# Autodesk Inventor assembly: RCP-2.0
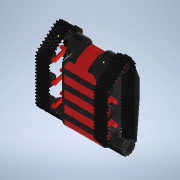
[picture p0: Inventor's stored thumbnail of the model, 180x180]
Saved by Autodesk Inventor 2020 (Build 240168000, 168)
## iProperties
Created: 2021-06-14
Part Number: RCP-2.0
Document SubType Name: Assembly
Designer: I_Love_U_Bogdan
Author: I_Love_U_Bogdan
## Documents named in this file (33)
- C:\Users\I_Love_U_Bogdan\Desktop\Work\Гусеничная платформа\RCP-2.0.iam
- C:\Users\I_Love_U_Bogdan\Desktop\Work\Гусеничная платформа\Корпус внутр.ipt
- C:\Users\I_Love_U_Bogdan\Desktop\Work\Гусеничная платформа\Корпус внутр2.ipt
- C:\Users\I_Love_U_Bogdan\Desktop\Work\Гусеничная платформа\Корпус.ipt
- C:\Users\I_Love_U_Bogdan\Desktop\Work\Гусеничная платформа\Корпус4.ipt
- C:\Users\I_Love_U_Bogdan\Desktop\Work\Гусеничная платформа\Перед-верх.ipt
- C:\Users\I_Love_U_Bogdan\Desktop\Work\Гусеничная платформа\СкреплениеКорпусПеред.ipt
- C:\Users\I_Love_U_Bogdan\Desktop\Work\Гусеничная платформа\РеброСкрепления.ipt
- C:\Users\I_Love_U_Bogdan\Desktop\Work\Гусеничная платформа\ВерхнийКрюк.ipt
- C:\Users\I_Love_U_Bogdan\Desktop\Work\Гусеничная платформа\РельсКрышки.ipt
- C:\Users\I_Love_U_Bogdan\Desktop\Work\Гусеничная платформа\Держатель каскада.ipt
- C:\Users\I_Love_U_Bogdan\Desktop\Work\Гусеничная платформа\запорные зубцы.ipt
- C:\Users\I_Love_U_Bogdan\Desktop\Work\Гусеничная платформа\Крышка.ipt
- C:\Users\I_Love_U_Bogdan\Desktop\Work\Гусеничная платформа\РучкаКрышки.ipt
- C:\Users\I_Love_U_Bogdan\Desktop\Work\Гусеничная платформа\Держатель каскада2.ipt
- C:\Users\I_Love_U_Bogdan\Desktop\Work\Гусеничная платформа\Пластина.ipt
- C:\Users\I_Love_U_Bogdan\Desktop\Work\Гусеничная платформа\ВедущееКолесо V2.ipt
- C:\Users\I_Love_U_Bogdan\Desktop\Work\Гусеничная платформа\Шаговик17.ipt
- C:\Users\I_Love_U_Bogdan\Desktop\Work\Гусеничная платформа\Муфта2.ipt
- C:\Users\I_Love_U_Bogdan\Desktop\Work\Гусеничная платформа\Втулка.ipt
- C:\Users\I_Love_U_Bogdan\Desktop\Work\Гусеничная платформа\ВнутрНат.ipt
- C:\Users\I_Love_U_Bogdan\Desktop\Work\Гусеничная платформа\ВнутрНатПр.ipt
- C:\Users\I_Love_U_Bogdan\Desktop\Work\Гусеничная платформа\ВнешНат.ipt
- C:\Users\I_Love_U_Bogdan\Desktop\Work\Гусеничная платформа\ВнешНатПр.ipt
- C:\Users\I_Love_U_Bogdan\Desktop\Work\Гусеничная платформа\ОпорныйКаток.ipt
- C:\Users\I_Love_U_Bogdan\Desktop\Work\Гусеничная платформа\ОпорныйКаток2.ipt
- C:\Users\I_Love_U_Bogdan\Desktop\Work\Гусеничная платформа\СкреплениеКатков.ipt
- C:\Users\I_Love_U_Bogdan\Desktop\Work\Гусеничная платформа\РычагОпорного.ipt
- C:\Users\I_Love_U_Bogdan\Desktop\Work\Гусеничная платформа\РычагОпорногоПравый.ipt
- C:\Users\I_Love_U_Bogdan\Desktop\Work\Гусеничная платформа\Надкрылок.ipt
- C:\Users\I_Love_U_Bogdan\Desktop\Work\Гусеничная платформа\НадкрылокПравый.ipt
- C:\Users\I_Love_U_Bogdan\Desktop\Work\Гусеничная платформа\Направляющая1.ipt
- C:\Users\I_Love_U_Bogdan\Desktop\Work\Гусеничная платформа\ТракV2.ipt
## Components (201 placed, 32 different names)
1. Шаговик17:1 — Совмещение:72, Совмещение:73, Совмещение:74, Совмещение:78, Совмещение:79
2. Шаговик17:2 — Совмещение:75, Совмещение:76, Совмещение:77, Совмещение:80, Совмещение:81
3. ВедущееКолесо V2:2 — Совмещение:82, Совмещение:86, Совмещение:87, Совмещение:195
4. Муфта2:1 — Совмещение:78, Совмещение:79, Совмещение:83, Совмещение:84, Совмещение:85, Угол:1
5. Муфта2:2 — Совмещение:80, Совмещение:81, Совмещение:82, Совмещение:86, Совмещение:87, Угол:2
6. ВедущееКолесо V2:3 — Совмещение:83, Совмещение:84, Совмещение:85, Совмещение:192
7. РычагОпорного:1 — Совмещение:116, Совмещение:117, Совмещение:128, Совмещение:171, Совмещение:175
8. РычагОпорного:2 — Совмещение:118, Совмещение:120, Совмещение:129, Совмещение:172, Совмещение:176
9. РычагОпорного:3 — Совмещение:119, Совмещение:121, Совмещение:130, Совмещение:173, Совмещение:177
10. РычагОпорногоПравый:1 — Совмещение:122, Совмещение:127, Совмещение:131, Совмещение:180, Совмещение:184
11. РычагОпорногоПравый:2 — Совмещение:123, Совмещение:126, Совмещение:132, Совмещение:179, Совмещение:183
12. РычагОпорногоПравый:3 — Совмещение:124, Совмещение:125, Совмещение:133, Совмещение:178, Совмещение:185
13. Надкрылок:1 — Совмещение:186, Совмещение:187, Совмещение:188
14. НадкрылокПравый:1 — Совмещение:189, Совмещение:190, Совмещение:191
15. Направляющая1:1 — Заподлицо:15, Заподлицо:16, Совмещение:194, Совмещение:196
16. Втулка:1 — Совмещение:91, Совмещение:92, Совмещение:93, Совмещение:95, Совмещение:99
17. Втулка:2 — Совмещение:88, Совмещение:89, Совмещение:90, Совмещение:94, Совмещение:98
18. ВнутрНат:1 — Совмещение:94, Совмещение:97, Совмещение:98, Совмещение:100, Совмещение:102
19. ВнутрНатПр:1 — Совмещение:95, Совмещение:96, Совмещение:99, Совмещение:101, Совмещение:103
20. ВнешНат:1 — Совмещение:100, Совмещение:102, Совмещение:170, Совмещение:174
21. ВнешНатПр:1 — Совмещение:101, Совмещение:103, Совмещение:181, Совмещение:182
22. ОпорныйКаток:1 — Совмещение:104, Совмещение:105, Совмещение:106, Совмещение:109
23. ОпорныйКаток2:1 — Совмещение:104, Совмещение:105, Совмещение:106, Совмещение:107, Совмещение:108, Совмещение:170, Совмещение:174
24. СкреплениеКатков:1 — Совмещение:107, Совмещение:108, Совмещение:109
25. ОпорныйКаток:2
26. ОпорныйКаток2:2 — Совмещение:171, Совмещение:175
27. СкреплениеКатков:2
28. ОпорныйКаток:3
29. ОпорныйКаток2:3 — Совмещение:172, Совмещение:176
30. СкреплениеКатков:3
31. ОпорныйКаток:4
32. ОпорныйКаток2:4 — Совмещение:173, Совмещение:177
33. СкреплениеКатков:4
34. ОпорныйКаток:5
35. ОпорныйКаток2:5 — Совмещение:178, Совмещение:185
36. СкреплениеКатков:5
37. ОпорныйКаток:6
38. ОпорныйКаток2:6 — Совмещение:179, Совмещение:183
39. СкреплениеКатков:6
40. ОпорныйКаток:7
41. ОпорныйКаток2:7 — Совмещение:180, Совмещение:184
42. СкреплениеКатков:7
43. ОпорныйКаток:8
44. ОпорныйКаток2:8 — Совмещение:181, Совмещение:182
45. СкреплениеКатков:8
46. Корпус внутр:1 — Совмещение:1, Совмещение:2, Совмещение:3, Совмещение:4, Заподлицо:1, Заподлицо:2, Совмещение:5, Заподлицо:3, Заподлицо:4, Совмещение:7, Заподлицо:7, Заподлицо:8, Совмещение:8, Совмещение:9, Совмещение:10
47. Корпус внутр2:1 — Совмещение:4, Заподлицо:1, Заподлицо:2, Совмещение:6, Заподлицо:5, Заподлицо:6, Совмещение:11, Совмещение:12, Совмещение:13, Совмещение:14, Совмещение:15, Совмещение:16, Совмещение:17, Совмещение:18, Совмещение:19, Совмещение:20
48. Корпус:1 — Совмещение:5, Заподлицо:3, Заподлицо:4, Совмещение:34, Совмещение:35, Совмещение:36, Заподлицо:13, Совмещение:71, Совмещение:72, Совмещение:73, Совмещение:74, Совмещение:88, Совмещение:89, Совмещение:90, Совмещение:97, Совмещение:116, Совмещение:117, Совмещение:118, Совмещение:119, Совмещение:120, Совмещение:121, Совмещение:128, Совмещение:129, Совмещение:130, Совмещение:186, Совмещение:187, Совмещение:188, Заподлицо:15, Заподлицо:16, Угол:1
49. Корпус4:1 — Совмещение:6, Заподлицо:5, Заподлицо:6, Совмещение:21, Совмещение:22, Совмещение:23, Совмещение:24, Совмещение:25, Совмещение:37, Совмещение:38, Совмещение:39, Совмещение:75, Совмещение:76, Совмещение:77, Совмещение:91, Совмещение:92, Совмещение:93, Совмещение:96, Совмещение:122, Совмещение:123, Совмещение:124, Совмещение:125, Совмещение:126, Совмещение:127, Совмещение:131, Совмещение:132, Совмещение:133, Совмещение:189, Совмещение:190, Совмещение:191, Угол:2
50. Перед-верх:1 — Совмещение:7, Заподлицо:7, Заподлицо:8, Совмещение:26, Совмещение:27, Совмещение:28, Совмещение:29, Совмещение:30, Совмещение:31, Совмещение:32, Совмещение:33, Заподлицо:9, Заподлицо:10, Заподлицо:11, Заподлицо:12, Заподлицо:14
51. СкреплениеКорпусПеред:1 — Совмещение:8, Совмещение:9, Совмещение:10
52. РеброСкрепления:1 — Совмещение:14, Совмещение:17, Совмещение:22
53. РеброСкрепления:2 — Совмещение:13, Совмещение:18, Совмещение:23
54. РеброСкрепления:3 — Совмещение:12, Совмещение:19, Совмещение:24
55. РеброСкрепления:4 — Совмещение:11, Совмещение:20, Совмещение:25
56. РеброСкрепления:5 — Совмещение:15, Совмещение:16, Совмещение:21
57. ВерхнийКрюк:1 — Совмещение:32, Совмещение:33, Заподлицо:9
58. ВерхнийКрюк:2 — Совмещение:28, Совмещение:29, Заподлицо:11
59. ВерхнийКрюк:3 — Совмещение:30, Совмещение:31, Заподлицо:10
60. ВерхнийКрюк:4 — Совмещение:26, Совмещение:27, Заподлицо:12
61. РельсКрышки:1 — Совмещение:34, Совмещение:35, Совмещение:36
62. РельсКрышки:2 — Совмещение:37, Совмещение:38, Совмещение:39
63. Держатель каскада:1 — Совмещение:43, Совмещение:44, Совмещение:45, Совмещение:48
64. запорные зубцы:1 — Совмещение:40, Совмещение:41, Совмещение:42
65. Крышка:1 — Совмещение:40, Совмещение:41, Совмещение:42, Совмещение:43, Совмещение:44, Совмещение:45, Совмещение:47, Совмещение:50, Совмещение:51, Совмещение:52, Совмещение:53, Совмещение:54, Совмещение:55, Совмещение:56, Совмещение:57, Совмещение:58, Совмещение:59, Совмещение:60, Совмещение:61, Совмещение:62, Совмещение:63, Совмещение:64, Совмещение:65, Совмещение:66, Совмещение:67, Совмещение:68, Совмещение:69, Совмещение:70, Заподлицо:13, Заподлицо:14, Совмещение:71
66. РучкаКрышки:1 — Совмещение:47, Совмещение:52
67. Держатель каскада2:1 — Совмещение:48, Совмещение:50, Совмещение:51
68. Пластина:1 — Совмещение:53, Совмещение:54, Совмещение:55
69. Пластина:2 — Совмещение:56, Совмещение:57, Совмещение:58
70. Пластина:3 — Совмещение:59, Совмещение:60, Совмещение:61
71. Пластина:4 — Совмещение:62, Совмещение:63, Совмещение:64
72. Пластина:5 — Совмещение:65, Совмещение:66, Совмещение:67
73. Пластина:6 — Совмещение:68, Совмещение:69, Совмещение:70
74. ТракV2:1 — Совмещение:192, Совмещение:194
75. ТракV2:2
76. ТракV2:3
77. ТракV2:4
78. ТракV2:5
79. ТракV2:6
80. ТракV2:7
81. ТракV2:8
82. ТракV2:9
83. ТракV2:10
84. ТракV2:11
85. ТракV2:12
86. ТракV2:13
87. ТракV2:14
88. ТракV2:15
89. ТракV2:16
90. ТракV2:17
91. ТракV2:18
92. ТракV2:19
93. ТракV2:20
94. ТракV2:21
95. ТракV2:22
96. ТракV2:23
97. ТракV2:24
98. ТракV2:25
99. ТракV2:26
100. ТракV2:27
101. ТракV2:28
102. ТракV2:29
103. ТракV2:30
104. ТракV2:31
105. ТракV2:32
106. ТракV2:33
107. ТракV2:34
108. ТракV2:35
109. ТракV2:36
110. ТракV2:37
111. ТракV2:38
112. ТракV2:39
113. ТракV2:40
114. ТракV2:41
115. ТракV2:42
116. ТракV2:43
117. ТракV2:44
118. ТракV2:45
119. ТракV2:46
120. ТракV2:47
121. ТракV2:48
122. ТракV2:49
123. ТракV2:50
124. ТракV2:51
125. ТракV2:52
126. ТракV2:53
127. ТракV2:54
128. ТракV2:55
129. ТракV2:56
130. ТракV2:57
131. ТракV2:58
132. ТракV2:59
133. ТракV2:60
134. ТракV2:61
135. ТракV2:62
136. ТракV2:63
137. ТракV2:64
138. ТракV2:65 — Совмещение:195, Совмещение:196
139. ТракV2:66
140. ТракV2:67
141. ТракV2:68
142. ТракV2:69
143. ТракV2:70
144. ТракV2:71
145. ТракV2:72
146. ТракV2:73
147. ТракV2:74
148. ТракV2:75
149. ТракV2:76
150. ТракV2:77
151. ТракV2:78
152. ТракV2:79
153. ТракV2:80
154. ТракV2:81
155. ТракV2:82
156. ТракV2:83
157. ТракV2:84
158. ТракV2:85
159. ТракV2:86
160. ТракV2:87
161. ТракV2:88
162. ТракV2:89
163. ТракV2:90
164. ТракV2:91
165. ТракV2:92
166. ТракV2:93
167. ТракV2:94
168. ТракV2:95
169. ТракV2:96
170. ТракV2:97
171. ТракV2:98
172. ТракV2:99
173. ТракV2:100
174. ТракV2:101
175. ТракV2:102
176. ТракV2:103
177. ТракV2:104
178. ТракV2:105
179. ТракV2:106
180. ТракV2:107
181. ТракV2:108
182. ТракV2:109
183. ТракV2:110
184. ТракV2:111
185. ТракV2:112
186. ТракV2:113
187. ТракV2:114
188. ТракV2:115
189. ТракV2:116
190. ТракV2:117
191. ТракV2:118
192. ТракV2:119
193. ТракV2:120
194. ТракV2:121
195. ТракV2:122
196. ТракV2:123
197. ТракV2:124
198. ТракV2:125
199. ТракV2:126
200. ТракV2:127
201. ТракV2:128
## Component patterns: ЛеваяГусеница (64 elements), ПраваяГусеница (64 elements)
## Relationships (211: Mate 193, Flush 16, Angle 2)
- Совмещение:1 [Mate]: Корпус внутр:1
- Совмещение:2 [Mate]: Корпус внутр:1
- Совмещение:3 [Mate] (100 mm): Корпус внутр:1
- Совмещение:4 [Mate]: Корпус внутр:1 ↔ Корпус внутр2:1
- Заподлицо:1 [Flush]: Корпус внутр:1 ↔ Корпус внутр2:1
- Заподлицо:2 [Flush]: Корпус внутр:1 ↔ Корпус внутр2:1
- Совмещение:5 [Mate]: Корпус внутр:1 ↔ Корпус:1
- Заподлицо:3 [Flush]: Корпус внутр:1 ↔ Корпус:1
- Заподлицо:4 [Flush]: Корпус внутр:1 ↔ Корпус:1
- Совмещение:6 [Mate]: Корпус внутр2:1 ↔ Корпус4:1
- Заподлицо:5 [Flush]: Корпус внутр2:1 ↔ Корпус4:1
- Заподлицо:6 [Flush]: Корпус внутр2:1 ↔ Корпус4:1
- Совмещение:7 [Mate]: Корпус внутр:1 ↔ Перед-верх:1
- Заподлицо:7 [Flush] (-1 mm): Корпус внутр:1 ↔ Перед-верх:1
- Заподлицо:8 [Flush]: Корпус внутр:1 ↔ Перед-верх:1
- Совмещение:8 [Mate]: Корпус внутр:1 ↔ СкреплениеКорпусПеред:1
- Совмещение:9 [Mate]: Корпус внутр:1 ↔ СкреплениеКорпусПеред:1
- Совмещение:10 [Mate]: Корпус внутр:1 ↔ СкреплениеКорпусПеред:1
- Совмещение:11 [Mate]: Корпус внутр2:1 ↔ РеброСкрепления:4
- Совмещение:12 [Mate]: Корпус внутр2:1 ↔ РеброСкрепления:3
- Совмещение:13 [Mate]: Корпус внутр2:1 ↔ РеброСкрепления:2
- Совмещение:14 [Mate]: Корпус внутр2:1 ↔ РеброСкрепления:1
- Совмещение:15 [Mate]: Корпус внутр2:1 ↔ РеброСкрепления:5
- Совмещение:16 [Mate] (0.1 mm): Корпус внутр2:1 ↔ РеброСкрепления:5
- Совмещение:17 [Mate] (0.1 mm): Корпус внутр2:1 ↔ РеброСкрепления:1
- Совмещение:18 [Mate] (0.1 mm): Корпус внутр2:1 ↔ РеброСкрепления:2
- Совмещение:19 [Mate] (0.1 mm): Корпус внутр2:1 ↔ РеброСкрепления:3
- Совмещение:20 [Mate] (0.1 mm): Корпус внутр2:1 ↔ РеброСкрепления:4
- Совмещение:21 [Mate] (0.1 mm): Корпус4:1 ↔ РеброСкрепления:5
- Совмещение:22 [Mate] (0.1 mm): Корпус4:1 ↔ РеброСкрепления:1
- Совмещение:23 [Mate] (0.1 mm): Корпус4:1 ↔ РеброСкрепления:2
- Совмещение:24 [Mate] (0.1 mm): Корпус4:1 ↔ РеброСкрепления:3
- Совмещение:25 [Mate] (0.1 mm): Корпус4:1 ↔ РеброСкрепления:4
- Совмещение:26 [Mate]: Перед-верх:1 ↔ ВерхнийКрюк:4
- Совмещение:27 [Mate]: Перед-верх:1 ↔ ВерхнийКрюк:4
- Совмещение:28 [Mate]: Перед-верх:1 ↔ ВерхнийКрюк:2
- Совмещение:29 [Mate]: Перед-верх:1 ↔ ВерхнийКрюк:2
- Совмещение:30 [Mate]: Перед-верх:1 ↔ ВерхнийКрюк:3
- Совмещение:31 [Mate]: Перед-верх:1 ↔ ВерхнийКрюк:3
- Совмещение:32 [Mate]: Перед-верх:1 ↔ ВерхнийКрюк:1
- Совмещение:33 [Mate]: Перед-верх:1 ↔ ВерхнийКрюк:1
- Заподлицо:9 [Flush] (-3 mm): Перед-верх:1 ↔ ВерхнийКрюк:1
- Заподлицо:10 [Flush] (-3 mm): Перед-верх:1 ↔ ВерхнийКрюк:3
- Заподлицо:11 [Flush] (-3 mm): Перед-верх:1 ↔ ВерхнийКрюк:2
- Заподлицо:12 [Flush] (-3 mm): Перед-верх:1 ↔ ВерхнийКрюк:4
- Совмещение:34 [Mate]: Корпус:1 ↔ РельсКрышки:1
- Совмещение:35 [Mate]: Корпус:1 ↔ РельсКрышки:1
- Совмещение:36 [Mate]: Корпус:1 ↔ РельсКрышки:1
- Совмещение:37 [Mate]: Корпус4:1 ↔ РельсКрышки:2
- Совмещение:38 [Mate]: Корпус4:1 ↔ РельсКрышки:2
- Совмещение:39 [Mate]: Корпус4:1 ↔ РельсКрышки:2
- Совмещение:40 [Mate]: запорные зубцы:1 ↔ Крышка:1
- Совмещение:41 [Mate]: запорные зубцы:1 ↔ Крышка:1
- Совмещение:42 [Mate]: запорные зубцы:1 ↔ Крышка:1
- Совмещение:43 [Mate] (0.17 mm): Держатель каскада:1 ↔ Крышка:1
- Совмещение:44 [Mate]: Держатель каскада:1 ↔ Крышка:1
- Совмещение:45 [Mate] (-70.8 mm): Держатель каскада:1 ↔ Крышка:1
- Совмещение:47 [Mate]: Крышка:1 ↔ РучкаКрышки:1
- Совмещение:48 [Mate]: Держатель каскада:1 ↔ Держатель каскада2:1
- Совмещение:50 [Mate]: Крышка:1 ↔ Держатель каскада2:1
- Совмещение:51 [Mate] (0.17 mm): Крышка:1 ↔ Держатель каскада2:1
- Совмещение:52 [Mate]: Крышка:1 ↔ РучкаКрышки:1
- Совмещение:53 [Mate]: Крышка:1 ↔ Пластина:1
- Совмещение:54 [Mate]: Крышка:1 ↔ Пластина:1
- Совмещение:55 [Mate] (0.4 mm): Крышка:1 ↔ Пластина:1
- Совмещение:56 [Mate]: Крышка:1 ↔ Пластина:2
- Совмещение:57 [Mate]: Крышка:1 ↔ Пластина:2
- Совмещение:58 [Mate] (0.4 mm): Крышка:1 ↔ Пластина:2
- Совмещение:59 [Mate]: Крышка:1 ↔ Пластина:3
- Совмещение:60 [Mate]: Крышка:1 ↔ Пластина:3
- Совмещение:61 [Mate] (0.4 mm): Крышка:1 ↔ Пластина:3
- Совмещение:62 [Mate]: Крышка:1 ↔ Пластина:4
- Совмещение:63 [Mate]: Крышка:1 ↔ Пластина:4
- Совмещение:64 [Mate] (0.4 mm): Крышка:1 ↔ Пластина:4
- Совмещение:65 [Mate]: Крышка:1 ↔ Пластина:5
- Совмещение:66 [Mate]: Крышка:1 ↔ Пластина:5
- Совмещение:67 [Mate] (0.4 mm): Крышка:1 ↔ Пластина:5
- Совмещение:68 [Mate]: Крышка:1 ↔ Пластина:6
- Совмещение:69 [Mate]: Крышка:1 ↔ Пластина:6
- Совмещение:70 [Mate] (0.4 mm): Крышка:1 ↔ Пластина:6
- Заподлицо:13 [Flush]: Корпус:1 ↔ Крышка:1
- Заподлицо:14 [Flush]: Перед-верх:1 ↔ Крышка:1
- Совмещение:71 [Mate] (0.2 mm): Корпус:1 ↔ Крышка:1
- Совмещение:72 [Mate]: Шаговик17:1 ↔ Корпус:1
- Совмещение:73 [Mate]: Шаговик17:1 ↔ Корпус:1
- Совмещение:74 [Mate]: Шаговик17:1 ↔ Корпус:1
- Совмещение:75 [Mate]: Шаговик17:2 ↔ Корпус4:1
- Совмещение:76 [Mate]: Шаговик17:2 ↔ Корпус4:1
- Совмещение:77 [Mate]: Шаговик17:2 ↔ Корпус4:1
- Совмещение:78 [Mate]: Шаговик17:1 ↔ Муфта2:1
- Совмещение:79 [Mate]: Шаговик17:1 ↔ Муфта2:1
- Совмещение:80 [Mate]: Шаговик17:2 ↔ Муфта2:2
- Совмещение:81 [Mate]: Шаговик17:2 ↔ Муфта2:2
- Совмещение:82 [Mate]: ВедущееКолесо V2:2 ↔ Муфта2:2
- Совмещение:83 [Mate]: Муфта2:1 ↔ ВедущееКолесо V2:3
- Совмещение:84 [Mate]: Муфта2:1 ↔ ВедущееКолесо V2:3
- Совмещение:85 [Mate]: Муфта2:1 ↔ ВедущееКолесо V2:3
- Совмещение:86 [Mate]: ВедущееКолесо V2:2 ↔ Муфта2:2
- Совмещение:87 [Mate]: ВедущееКолесо V2:2 ↔ Муфта2:2
- Совмещение:88 [Mate]: Втулка:2 ↔ Корпус:1
- Совмещение:89 [Mate] (0.2 mm): Втулка:2 ↔ Корпус:1
- Совмещение:90 [Mate]: Втулка:2 ↔ Корпус:1
- Совмещение:91 [Mate]: Втулка:1 ↔ Корпус4:1
- Совмещение:92 [Mate] (0.2 mm): Втулка:1 ↔ Корпус4:1
- Совмещение:93 [Mate]: Втулка:1 ↔ Корпус4:1
- Совмещение:94 [Mate]: Втулка:2 ↔ ВнутрНат:1
- Совмещение:95 [Mate]: Втулка:1 ↔ ВнутрНатПр:1
- Совмещение:96 [Mate] (4 mm): ВнутрНатПр:1 ↔ Корпус4:1
- Совмещение:97 [Mate] (4 mm): ВнутрНат:1 ↔ Корпус:1
- Совмещение:98 [Mate]: Втулка:2 ↔ ВнутрНат:1
- Совмещение:99 [Mate]: Втулка:1 ↔ ВнутрНатПр:1
- Совмещение:100 [Mate]: ВнутрНат:1 ↔ ВнешНат:1
- Совмещение:101 [Mate]: ВнутрНатПр:1 ↔ ВнешНатПр:1
- Совмещение:102 [Mate]: ВнутрНат:1 ↔ ВнешНат:1
- Совмещение:103 [Mate]: ВнутрНатПр:1 ↔ ВнешНатПр:1
- Совмещение:104 [Mate]: ОпорныйКаток:1 ↔ ОпорныйКаток2:1
- Совмещение:105 [Mate]: ОпорныйКаток:1 ↔ ОпорныйКаток2:1
- Совмещение:106 [Mate]: ОпорныйКаток:1 ↔ ОпорныйКаток2:1
- Совмещение:107 [Mate]: ОпорныйКаток2:1 ↔ СкреплениеКатков:1
- Совмещение:108 [Mate]: ОпорныйКаток2:1 ↔ СкреплениеКатков:1
- Совмещение:109 [Mate]: ОпорныйКаток:1 ↔ СкреплениеКатков:1
- [Mate]: ОпорныйКаток:2 ↔ ОпорныйКаток2:2
- [Mate]: ОпорныйКаток:2 ↔ ОпорныйКаток2:2
- [Mate]: ОпорныйКаток:2 ↔ ОпорныйКаток2:2
- [Mate]: ОпорныйКаток2:2 ↔ СкреплениеКатков:2
- [Mate]: ОпорныйКаток2:2 ↔ СкреплениеКатков:2
- [Mate]: ОпорныйКаток:2 ↔ СкреплениеКатков:2
- Совмещение:116 [Mate]: РычагОпорного:1 ↔ Корпус:1
- Совмещение:117 [Mate] (1 mm): РычагОпорного:1 ↔ Корпус:1
- Совмещение:118 [Mate]: РычагОпорного:2 ↔ Корпус:1
- Совмещение:119 [Mate]: РычагОпорного:3 ↔ Корпус:1
- Совмещение:120 [Mate] (2 mm): РычагОпорного:2 ↔ Корпус:1
- Совмещение:121 [Mate] (2 mm): РычагОпорного:3 ↔ Корпус:1
- Совмещение:122 [Mate]: РычагОпорногоПравый:1 ↔ Корпус4:1
- Совмещение:123 [Mate]: РычагОпорногоПравый:2 ↔ Корпус4:1
- Совмещение:124 [Mate]: РычагОпорногоПравый:3 ↔ Корпус4:1
- Совмещение:125 [Mate] (2 mm): РычагОпорногоПравый:3 ↔ Корпус4:1
- Совмещение:126 [Mate] (2 mm): РычагОпорногоПравый:2 ↔ Корпус4:1
- Совмещение:127 [Mate] (2 mm): РычагОпорногоПравый:1 ↔ Корпус4:1
- Совмещение:128 [Mate]: РычагОпорного:1 ↔ Корпус:1
- Совмещение:129 [Mate]: РычагОпорного:2 ↔ Корпус:1
- Совмещение:130 [Mate]: РычагОпорного:3 ↔ Корпус:1
- Совмещение:131 [Mate]: РычагОпорногоПравый:1 ↔ Корпус4:1
- Совмещение:132 [Mate]: РычагОпорногоПравый:2 ↔ Корпус4:1
- Совмещение:133 [Mate]: РычагОпорногоПравый:3 ↔ Корпус4:1
- [Mate]: ОпорныйКаток:3 ↔ ОпорныйКаток2:3
- [Mate]: ОпорныйКаток:3 ↔ ОпорныйКаток2:3
- [Mate]: ОпорныйКаток:3 ↔ ОпорныйКаток2:3
- [Mate]: ОпорныйКаток2:3 ↔ СкреплениеКатков:3
- [Mate]: ОпорныйКаток2:3 ↔ СкреплениеКатков:3
- [Mate]: ОпорныйКаток:3 ↔ СкреплениеКатков:3
- [Mate]: ОпорныйКаток:4 ↔ ОпорныйКаток2:4
- [Mate]: ОпорныйКаток:4 ↔ ОпорныйКаток2:4
- [Mate]: ОпорныйКаток:4 ↔ ОпорныйКаток2:4
- [Mate]: ОпорныйКаток2:4 ↔ СкреплениеКатков:4
- [Mate]: ОпорныйКаток2:4 ↔ СкреплениеКатков:4
- [Mate]: ОпорныйКаток:4 ↔ СкреплениеКатков:4
- [Mate]: ОпорныйКаток:5 ↔ ОпорныйКаток2:5
- [Mate]: ОпорныйКаток:5 ↔ ОпорныйКаток2:5
- [Mate]: ОпорныйКаток:5 ↔ ОпорныйКаток2:5
- [Mate]: ОпорныйКаток2:5 ↔ СкреплениеКатков:5
- [Mate]: ОпорныйКаток2:5 ↔ СкреплениеКатков:5
- [Mate]: ОпорныйКаток:5 ↔ СкреплениеКатков:5
- [Mate]: ОпорныйКаток:6 ↔ ОпорныйКаток2:6
- [Mate]: ОпорныйКаток:6 ↔ ОпорныйКаток2:6
- [Mate]: ОпорныйКаток:6 ↔ ОпорныйКаток2:6
- [Mate]: ОпорныйКаток2:6 ↔ СкреплениеКатков:6
- [Mate]: ОпорныйКаток2:6 ↔ СкреплениеКатков:6
- [Mate]: ОпорныйКаток:6 ↔ СкреплениеКатков:6
- [Mate]: ОпорныйКаток:7 ↔ ОпорныйКаток2:7
- [Mate]: ОпорныйКаток:7 ↔ ОпорныйКаток2:7
- [Mate]: ОпорныйКаток:7 ↔ ОпорныйКаток2:7
- [Mate]: ОпорныйКаток2:7 ↔ СкреплениеКатков:7
- [Mate]: ОпорныйКаток2:7 ↔ СкреплениеКатков:7
- [Mate]: ОпорныйКаток:7 ↔ СкреплениеКатков:7
- [Mate]: ОпорныйКаток:8 ↔ ОпорныйКаток2:8
- [Mate]: ОпорныйКаток:8 ↔ ОпорныйКаток2:8
- [Mate]: ОпорныйКаток:8 ↔ ОпорныйКаток2:8
- [Mate]: ОпорныйКаток2:8 ↔ СкреплениеКатков:8
- [Mate]: ОпорныйКаток2:8 ↔ СкреплениеКатков:8
- [Mate]: ОпорныйКаток:8 ↔ СкреплениеКатков:8
- Совмещение:170 [Mate]: ВнешНат:1 ↔ ОпорныйКаток2:1
- Совмещение:171 [Mate]: РычагОпорного:1 ↔ ОпорныйКаток2:2
- Совмещение:172 [Mate]: РычагОпорного:2 ↔ ОпорныйКаток2:3
- Совмещение:173 [Mate]: РычагОпорного:3 ↔ ОпорныйКаток2:4
- Совмещение:174 [Mate] (0.2 mm): ВнешНат:1 ↔ ОпорныйКаток2:1
- Совмещение:175 [Mate] (0.2 mm): РычагОпорного:1 ↔ ОпорныйКаток2:2
- Совмещение:176 [Mate] (0.2 mm): РычагОпорного:2 ↔ ОпорныйКаток2:3
- Совмещение:177 [Mate] (0.2 mm): РычагОпорного:3 ↔ ОпорныйКаток2:4
- Совмещение:178 [Mate]: РычагОпорногоПравый:3 ↔ ОпорныйКаток2:5
- Совмещение:179 [Mate]: РычагОпорногоПравый:2 ↔ ОпорныйКаток2:6
- Совмещение:180 [Mate]: РычагОпорногоПравый:1 ↔ ОпорныйКаток2:7
- Совмещение:181 [Mate]: ВнешНатПр:1 ↔ ОпорныйКаток2:8
- Совмещение:182 [Mate] (0.2 mm): ВнешНатПр:1 ↔ ОпорныйКаток2:8
- Совмещение:183 [Mate] (0.2 mm): РычагОпорногоПравый:2 ↔ ОпорныйКаток2:6
- Совмещение:184 [Mate] (0.2 mm): РычагОпорногоПравый:1 ↔ ОпорныйКаток2:7
- Совмещение:185 [Mate] (0.2 mm): РычагОпорногоПравый:3 ↔ ОпорныйКаток2:5
- Совмещение:186 [Mate]: Надкрылок:1 ↔ Корпус:1
- Совмещение:187 [Mate]: Надкрылок:1 ↔ Корпус:1
- Совмещение:188 [Mate]: Надкрылок:1 ↔ Корпус:1
- Совмещение:189 [Mate]: НадкрылокПравый:1 ↔ Корпус4:1
- Совмещение:190 [Mate]: НадкрылокПравый:1 ↔ Корпус4:1
- Совмещение:191 [Mate]: НадкрылокПравый:1 ↔ Корпус4:1
- Заподлицо:15 [Flush]: Направляющая1:1 ↔ Корпус:1
- Заподлицо:16 [Flush]: Направляющая1:1 ↔ Корпус:1
- Совмещение:192 [Mate] (0.4 mm): ВедущееКолесо V2:3 ↔ ТракV2:1
- Совмещение:194 [Mate] (2 mm): Направляющая1:1 ↔ ТракV2:1
- Угол:1 [Angle] (45 deg): Муфта2:1 ↔ Корпус:1
- Угол:2 [Angle] (0 deg): Муфта2:2 ↔ Корпус4:1
- Совмещение:195 [Mate] (0.4 mm): ВедущееКолесо V2:2 ↔ ТракV2:65
- Совмещение:196 [Mate] (2 mm): Направляющая1:1 ↔ ТракV2:65
## Named parameters: d126_d120 = 0 mm, d127_d121 = 0 mm, d128_d122 = 0 mm, d129_d123 = 0 mm, d130_d124 = 0 mm, d131_d125 = 0 mm, d150_d126_d120 = 0 mm, d151_d127_d121 = 0 mm, d152_d128_d122 = 0 mm, d153_d129_d123 = 0 mm, d154_d130_d124 = 0 mm, d155_d131_d125 = 0 mm, d156_d126_d120 = 0 mm, d157_d127_d121 = 0 mm, d158_d128_d122 = 0 mm, d159_d129_d123 = 0 mm, d160_d130_d124 = 0 mm, d161_d131_d125 = 0 mm, d162_d126_d120 = 0 mm, d163_d127_d121 = 0 mm, d164_d128_d122 = 0 mm, d165_d129_d123 = 0 mm, d166_d130_d124 = 0 mm, d167_d131_d125 = 0 mm, d168_d126_d120 = 0 mm, d169_d127_d121 = 0 mm, d170_d128_d122 = 0 mm, d171_d129_d123 = 0 mm, d172_d130_d124 = 0 mm, d173_d131_d125 = 0 mm, d174_d126_d120 = 0 mm, d175_d127_d121 = 0 mm, d176_d128_d122 = 0 mm, d177_d129_d123 = 0 mm, d178_d130_d124 = 0 mm, d179_d131_d125 = 0 mm, d180_d126_d120 = 0 mm, d181_d127_d121 = 0 mm, d182_d128_d122 = 0 mm, d183_d129_d123 = 0 mm, d184_d130_d124 = 0 mm, d185_d131_d125 = 0 mm
